# Autodesk Inventor assembly: z axis
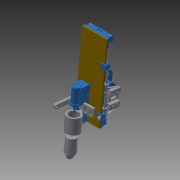
[picture p0: Inventor's stored thumbnail of the model, 180x180]
Saved by Autodesk Inventor 2013 SP2 (Build 170200200, 200)
## iProperties
Created: 2017-05-18
Part Number: z axis
Document SubType Name: Assembly
Designer: Herman de Vries
Author: Herman de Vries
## Documents named in this file (21)
- C:\Users\hdv\Dropbox\Projects\Inventor\PaintBot_3\z_axis\z axis.iam
- C:\Users\hdv\Dropbox\Projects\Inventor\PaintBot_3\z_axis\z endcap.ipt
- C:\Users\hdv\Dropbox\Projects\Inventor\PaintBot_3\z_axis\rod 3x150mm.ipt
- C:\Users\hdv\Dropbox\Projects\Inventor\PaintBot_3\z_axis\bearing linear 3x7x10mm.ipt
- C:\Users\hdv\Dropbox\Projects\Inventor\PaintBot_3\z_axis\L bracket.ipt
- C:\Users\hdv\Dropbox\Projects\Inventor\PaintBot_3\z_axis\bearing bed2.ipt
- C:\Users\hdv\Dropbox\Projects\Inventor\PaintBot_3\gear belt.ipt
- C:\Users\hdv\Dropbox\Projects\Inventor\PaintBot_3\z_axis\bearing flanged 10x3x4mm.ipt
- C:\Users\hdv\Dropbox\Projects\Inventor\parts\P-BD000007 - Screw M3x8mm Pozi SS ISO7045(Z).ipt
- C:\Users\hdv\Dropbox\Projects\Inventor\parts\Nut M3 Hex SS.ipt
- C:\Users\hdv\Dropbox\Projects\Inventor\parts\P-BD000036-Screw M3x20mm Hex Socket Head Cap SS ISO 4762.ipt
- C:\Users\hdv\Dropbox\Projects\Inventor\PaintBot_3\NEMA14.ipt
- C:\Users\hdv\Dropbox\Projects\Inventor\PaintBot_3\lever switch 20x10x6.ipt
- C:\Users\hdv\Dropbox\Projects\Inventor\PaintBot_3\Paint brush Platform.ipt
- C:\Users\hdv\Dropbox\Projects\Inventor\PaintBot_3\end limit holder.ipt
- C:\Users\hdv\Dropbox\Projects\Inventor\PaintBot_3\End stop clip.ipt
- C:\Users\hdv\Dropbox\Projects\Inventor\parts\P-BD000010-Screw M3x16mm Hex Socket Head Cap SS.ipt
- C:\Users\hdv\Dropbox\Projects\Inventor\PaintBot_3\Solinoid.ipt
- C:\Users\hdv\Dropbox\Projects\Inventor\PaintBot_3\Brush holder\brush holder assy v5.iam
- C:\Users\hdv\Dropbox\Projects\Inventor\PaintBot_3\Brush holder\Solinoid holder v5.ipt
- C:\Users\hdv\Dropbox\Projects\Inventor\PaintBot_3\Brush holder\switch bracket v5.1.ipt
## Components (32 placed, 20 different names)
1. z endcap:1 — Insert:1, Insert:2, Mate:33
2. z endcap:2 — Insert:3, Insert:4, Mate:22, Flush:22, Flush:23, Mate:34
3. rod 3x150mm:1 — Insert:1, Insert:3, Mate:1, Mate:3
4. rod 3x150mm:2 — Insert:2, Insert:4, Mate:2, Mate:4
5. bearing linear 3x7x10mm:1 — Mate:3, Mate:7, Flush:4
6. bearing linear 3x7x10mm:2 — Mate:4, Flush:13, Mate:14, Flush:14
7. bearing linear 3x7x10mm:3 — Mate:2, Flush:16
8. bearing linear 3x7x10mm:4 — Mate:1, Flush:7
9. L bracket:1 — Mate:9, Flush:12, Mate:11, Mate:13, Flush:17, Mate:19, Mate:20, Insert:5, Insert:7, Insert:8, Flush:18, Flush:19, Insert:9, Flush:26
10. bearing bed2:1 — Flush:13, Mate:13, Mate:14, Flush:14, Flush:15, Flush:16
11. bearing bed2:2 — Mate:7, Flush:4, Flush:7, Mate:9, Flush:12, Flush:15, Flush:17, Insert:6, Mate:27
12. NEMA14:1 — Mate:11, Mate:12, Flush:18, Flush:19, Flush:27
13. gear belt:1 — Mate:12, Flush:27
14. bearing flanged 10x3x4mm:1 — Mate:17, Mate:18, Mate:19, Mate:20
15. bearing flanged 10x3x4mm:2 — Mate:17, Mate:18
16. P-BD000007 - Screw M3x8mm Pozi SS ISO7045(Z):1 — Insert:6
17. DIN 934 - replaced by DIN EN 24032/28673/28674 M4:1 — Insert:5
18. DIN 934 - replaced by DIN EN 24032/28673/28674 M4:3 — Insert:7
19. P-BD000036 - Screw M3x20mm Hex Socket Head Cap SS:1 — Insert:8
20. bearing flanged 10x3x4mm:3 — Insert:9, Insert:10
21. bearing flanged 10x3x4mm:4 — Insert:10
22. lever switch 20x10x6:1 — Flush:24, Flush:25, Mate:28, Mate:29
23. Paint brush Platform:1 — Mate:22, Flush:22, Flush:23, Mate:31, Mate:32, Flush:28, Flush:29, Mate:37, Flush:32, Mate:40, Flush:33
24. lever switch 20x10x6:2 — Flush:24, Flush:25, Mate:30
25. end limit holder:1 — Mate:27, Mate:28, Mate:29, Mate:30, Flush:26
26. End stop clip:1 — Mate:31, Flush:29, Mate:34
27. End stop clip:2 — Mate:32, Flush:28, Insert:11, Mate:33
28. P-BD000010 - Screw M3x16mm Hex Socket Head Cap SS:1 — Insert:11
29. Solinoid:1 — Mate:38, Mate:39
30. Solinoid holder v5:1 — Mate:37, Mate:38, Mate:39, Flush:32, Mate:41, Flush:33, Insert:12
31. brush holder assy v5:1 [sub-assembly] — Mate:40, Mate:41
32. switch bracket v5.1:1 — Insert:12
## Relationships (61: Mate 29, Flush 20, Insert 12)
- Insert:1: z endcap:1 ↔ rod 3x150mm:1
- Insert:2: z endcap:1 ↔ rod 3x150mm:2
- Insert:3: z endcap:2 ↔ rod 3x150mm:1
- Insert:4: z endcap:2 ↔ rod 3x150mm:2
- Mate:1: rod 3x150mm:1 ↔ bearing linear 3x7x10mm:4
- Mate:2: rod 3x150mm:2 ↔ bearing linear 3x7x10mm:3
- Mate:3: rod 3x150mm:1 ↔ bearing linear 3x7x10mm:1
- Mate:4: rod 3x150mm:2 ↔ bearing linear 3x7x10mm:2
- Mate:7: bearing linear 3x7x10mm:1 ↔ bearing bed2:2
- Flush:4: bearing linear 3x7x10mm:1 ↔ bearing bed2:2
- Flush:7: bearing linear 3x7x10mm:4 ↔ bearing bed2:2
- Mate:9: L bracket:1 ↔ bearing bed2:2
- Flush:12: L bracket:1 ↔ bearing bed2:2
- Mate:11: L bracket:1 ↔ NEMA14:1
- Mate:12: NEMA14:1 ↔ gear belt:1
- Flush:13: bearing linear 3x7x10mm:2 ↔ bearing bed2:1
- Mate:13: L bracket:1 ↔ bearing bed2:1
- Mate:14: bearing linear 3x7x10mm:2 ↔ bearing bed2:1
- Flush:14: bearing linear 3x7x10mm:2 ↔ bearing bed2:1
- Flush:15: bearing bed2:1 ↔ bearing bed2:2
- Flush:16: bearing linear 3x7x10mm:3 ↔ bearing bed2:1
- Flush:17 (-5 mm): L bracket:1 ↔ bearing bed2:2
- Mate:17 (0.2 mm): bearing flanged 10x3x4mm:1 ↔ bearing flanged 10x3x4mm:2
- Mate:18: bearing flanged 10x3x4mm:1 ↔ bearing flanged 10x3x4mm:2
- Mate:19: L bracket:1 ↔ bearing flanged 10x3x4mm:1
- Mate:20 (0.8 mm): L bracket:1 ↔ bearing flanged 10x3x4mm:1
- Insert:5: L bracket:1 ↔ DIN 934 - replaced by DIN EN 24032/28673/28674 M4:1
- Insert:6: bearing bed2:2 ↔ P-BD000007 - Screw M3x8mm Pozi SS ISO7045(Z):1
- Insert:7: L bracket:1 ↔ DIN 934 - replaced by DIN EN 24032/28673/28674 M4:3
- Insert:8: L bracket:1 ↔ P-BD000036 - Screw M3x20mm Hex Socket Head Cap SS:1
- Flush:18 (12 mm): L bracket:1 ↔ NEMA14:1
- Flush:19 (2.5 mm): L bracket:1 ↔ NEMA14:1
- Insert:9 (0.2 mm): L bracket:1 ↔ bearing flanged 10x3x4mm:3
- Insert:10 (0.2 mm): bearing flanged 10x3x4mm:3 ↔ bearing flanged 10x3x4mm:4
- Mate:22: z endcap:2 ↔ Paint brush Platform:1
- Flush:22: z endcap:2 ↔ Paint brush Platform:1
- Flush:23: z endcap:2 ↔ Paint brush Platform:1
- Flush:24: lever switch 20x10x6:1 ↔ lever switch 20x10x6:2
- Flush:25: lever switch 20x10x6:1 ↔ lever switch 20x10x6:2
- [Mate]: L bracket:1 ↔ end limit holder:1
- Mate:27: bearing bed2:2 ↔ end limit holder:1
- Mate:28: lever switch 20x10x6:1 ↔ end limit holder:1
- Mate:29: lever switch 20x10x6:1 ↔ end limit holder:1
- Mate:30: lever switch 20x10x6:2 ↔ end limit holder:1
- Flush:26 (14 mm): L bracket:1 ↔ end limit holder:1
- Flush:27 (6 mm): NEMA14:1 ↔ gear belt:1
- Mate:31: Paint brush Platform:1 ↔ End stop clip:1
- Mate:32: Paint brush Platform:1 ↔ End stop clip:2
- Flush:28 (-5 mm): Paint brush Platform:1 ↔ End stop clip:2
- Flush:29 (-5 mm): Paint brush Platform:1 ↔ End stop clip:1
- Insert:11: End stop clip:2 ↔ P-BD000010 - Screw M3x16mm Hex Socket Head Cap SS:1
- Mate:33 (1 mm): z endcap:1 ↔ End stop clip:2
- Mate:34 (25 mm): z endcap:2 ↔ End stop clip:1
- Mate:37: Paint brush Platform:1 ↔ Solinoid holder v5:1
- Mate:38: Solinoid:1 ↔ Solinoid holder v5:1
- Mate:39: Solinoid:1 ↔ Solinoid holder v5:1
- Flush:32 (7 mm): Paint brush Platform:1 ↔ Solinoid holder v5:1
- Mate:40: Paint brush Platform:1 ↔ brush holder assy v5:1
- Mate:41: Solinoid holder v5:1 ↔ brush holder assy v5:1
- Flush:33: Paint brush Platform:1 ↔ Solinoid holder v5:1
- Insert:12: Solinoid holder v5:1 ↔ switch bracket v5.1:1
